# Autodesk Inventor assembly: soporte-botella
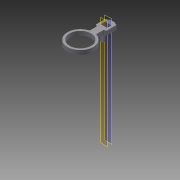
[picture p0: Inventor's stored thumbnail of the model, 180x180]
Saved by Autodesk Inventor 2015 SP1 (Build 190203100, 203)
## iProperties
Created: 2015-07-05
Part Number: soporte-botella
Document SubType Name: Assembly
Designer: Javier
Author: Javier
## Documents named in this file (4)
- D:\Dropbox\3dprint\riego\soporte-botella.iam
- D:\Dropbox\3dprint\riego\base_botella.ipt
- D:\Dropbox\3dprint\riego\brazo_botella.ipt
- D:\Dropbox\3dprint\riego\soporte-sujeccion-botella.ipt
## Components (3 placed, 3 different names)
1. base_botella:1 — Nivelación:1, Nivelación:2
2. brazo_botella:1 — Nivelación:1, Nivelación:2, Nivelación:3, Nivelación:4, Nivelación:5
3. soporte-sujeccion-botella:1 — Nivelación:3, Nivelación:4, Nivelación:5
## Relationships (5: Flush 5)
- Nivelación:1 [Flush]: base_botella:1 ↔ brazo_botella:1
- Nivelación:2 [Flush]: base_botella:1 ↔ brazo_botella:1
- Nivelación:3 [Flush]: brazo_botella:1 ↔ soporte-sujeccion-botella:1
- Nivelación:4 [Flush]: brazo_botella:1 ↔ soporte-sujeccion-botella:1
- Nivelación:5 [Flush]: brazo_botella:1 ↔ soporte-sujeccion-botella:1
